# Autodesk Inventor assembly: assembly.rev5
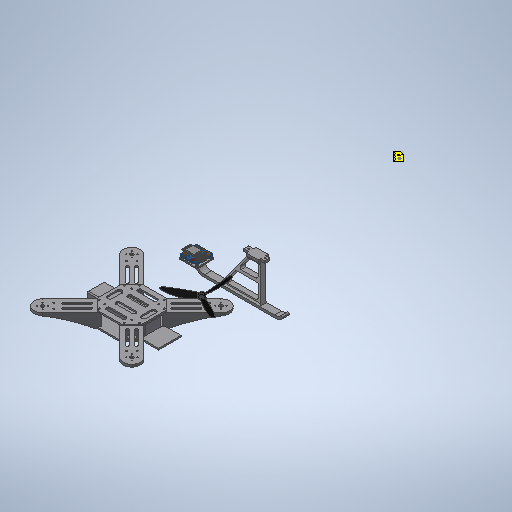
[picture p0: Inventor's stored thumbnail of the model, 512x512]
Saved by Autodesk Inventor 2025.2 (Build 292293000, 293)
## iProperties
Created: 2016-03-08
Part Number: assembly.rev5
Document SubType Name: Assembly
Designer: 200288284
Author: 200288284
## Documents named in this file (10)
- D:\UAV\esp drone\diy-drone\mechanical\新版 4.5\完整体.iam
- D:\UAV\esp drone\diy-drone\mechanical\新版 4.5\电池.ipt
- D:\UAV\esp drone\diy-drone\mechanical\新版 4.5\底板.ipt
- D:\UAV\esp drone\diy-drone\mechanical\新版 4.5\新起落架.ipt
- D:\UAV\esp drone\diy-drone\mechanical\新版 4.5\机臂.ipt
- D:\UAV\esp drone\diy-drone\mechanical\新版 4.5\上板.ipt
- D:\UAV\esp drone\diy-drone\mechanical\新版 4.5\5045 CW.ipt
- D:\UAV\esp drone\diy-drone\mechanical\新版 4.5\飞控板\飞控板\飞控板.ipt
- D:\UAV\esp drone\diy-drone\mechanical\新版 4.5\飞控盒\飞控盒.iam
- D:\UAV\esp drone\diy-drone\mechanical\新版 4.5\下板.ipt
## Components (12 placed, 9 different names)
1. 底板:1
2. 电池:2 — 配合:15, 表面齐平:1
3. 新起落架:1 — 配合:32
4. 机臂:1 — 配合:20, 配合:21, 配合:22, 配合:31
5. 上板:1 — 配合:10, 角度:1, 配合:11, 配合:15, 配合:16, 配合:17, 配合:18, 配合:20, 配合:21, 配合:22, 配合:23, 配合:24, 配合:25, 配合:26, 配合:27, 配合:28, 表面齐平:1
6. 5045 CW:1
7. 飞控板:1 — 配合:12, 配合:13, 配合:14
8. 飞控盒:1 [sub-assembly] — 配合:11, 配合:12, 配合:13, 配合:14
9. 机臂:2 — 配合:16, 配合:17, 配合:18
10. 机臂:3 — 配合:23, 配合:24, 配合:25, 配合:29, 配合:30
11. 机臂:4 — 配合:26, 配合:27, 配合:28
12. 下板:1 — 配合:29, 配合:30, 配合:31, 配合:32
## Relationships (24: Mate 22, Angle 1, Flush 1)
- 配合:10 [Mate]: 上板:1
- 角度:1 [Angle] (0 deg): 上板:1
- 配合:11 [Mate]: 上板:1 ↔ 飞控盒:1
- 配合:12 [Mate]: 飞控板:1 ↔ 飞控盒:1
- 配合:13 [Mate]: 飞控板:1 ↔ 飞控盒:1
- 配合:14 [Mate]: 飞控板:1 ↔ 飞控盒:1
- 配合:15 [Mate]: 电池:2 ↔ 上板:1
- 配合:16 [Mate]: 上板:1 ↔ 机臂:2
- 配合:17 [Mate]: 上板:1 ↔ 机臂:2
- 配合:18 [Mate]: 上板:1 ↔ 机臂:2
- 配合:20 [Mate]: 机臂:1 ↔ 上板:1
- 配合:21 [Mate]: 机臂:1 ↔ 上板:1
- 配合:22 [Mate]: 机臂:1 ↔ 上板:1
- 配合:23 [Mate]: 上板:1 ↔ 机臂:3
- 配合:24 [Mate]: 上板:1 ↔ 机臂:3
- 配合:25 [Mate]: 上板:1 ↔ 机臂:3
- 配合:26 [Mate]: 上板:1 ↔ 机臂:4
- 配合:27 [Mate]: 上板:1 ↔ 机臂:4
- 配合:28 [Mate]: 上板:1 ↔ 机臂:4
- 表面齐平:1 [Flush]: 电池:2 ↔ 上板:1
- 配合:29 [Mate]: 机臂:3 ↔ 下板:1
- 配合:30 [Mate]: 机臂:3 ↔ 下板:1
- 配合:31 [Mate]: 机臂:1 ↔ 下板:1
- 配合:32 [Mate]: 新起落架:1 ↔ 下板:1
